# Autodesk Inventor assembly: Ensamble eje + chaveta
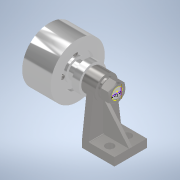
[picture p0: Inventor's stored thumbnail of the model, 180x180]
Saved by Autodesk Inventor 2021 (Build 250183000, 183)
## iProperties
Created: 2021-01-10
Part Number: Ensamble eje + chaveta
Document SubType Name: Assembly
Designer: dieku
Author: dieku
## Documents named in this file (3)
- C:\Users\dieku\Documents\GitHub\tallerDibujoIngenieria\Ensambles\Ensamble eje + chaveta.iam
- C:\Users\dieku\Documents\GitHub\tallerDibujoIngenieria\Ensambles\Ensamble chaveta exterior mas tensor polea.iam
- C:\Users\dieku\Documents\GitHub\tallerDibujoIngenieria\Ensambles\Ensamble tensor + eje.iam
## Components (2 placed, 2 different names)
1. Ensamble chaveta exterior mas tensor polea:1 [sub-assembly] — Insert:1
2. Ensamble tensor + eje:1 [sub-assembly] — Insert:1
## Relationships (1: Insert 1)
- Insert:1: Ensamble chaveta exterior mas tensor polea:1 ↔ Ensamble tensor + eje:1
